# Autodesk Inventor assembly: Flat_Panel
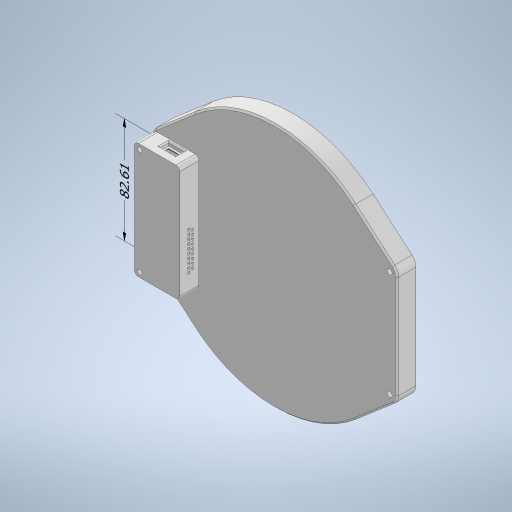
[picture p0: Inventor's stored thumbnail of the model, 512x512]
Saved by Autodesk Inventor 2024 (Build 280153000, 153)
## iProperties
Created: 2024-01-24
Part Number: Flat_Panel
Description: FreeCAD Model
Document SubType Name: Assembly
Designer: crow
Authority: Unknown
Sending System: FreeCAD
Preprocessor: Open CASCADE STEP processor 7.6
Title: Open CASCADE Shape Model
Author: Author
## Documents named in this file (6)
- C:\Users\crow\Documents\Github\EspFlatPanel\3d_print\inventor_Flat_Panel\FreeCAD_Model-Flat_Panel.iam
- C:\Users\crow\Documents\Github\EspFlatPanel\3d_print\inventor_Flat_Panel\Body.ipt
- C:\Users\crow\Documents\Github\EspFlatPanel\3d_print\inventor_Flat_Panel\Front.ipt
- C:\Users\crow\Documents\Github\EspFlatPanel\3d_print\inventor_Flat_Panel\Spacer.ipt
- C:\Users\crow\Documents\Github\EspFlatPanel\3d_print\inventor_Flat_Panel\Cover.ipt
- C:\Users\crow\Documents\Github\EspFlatPanel\3d_print\inventor_Flat_Panel\assembly_esp.iam
## Components (5 placed, 5 different names)
1. 5 — Rigid:2
2. 6
3. 7
4. 8
5. assembly_esp:1 [sub-assembly] — Rigid:2
## Relationships (1: WeldJoint 1)
- Rigid:2 [WeldJoint]: 5 ↔ assembly_esp:1
